# Autodesk Inventor assembly: BaseBoard
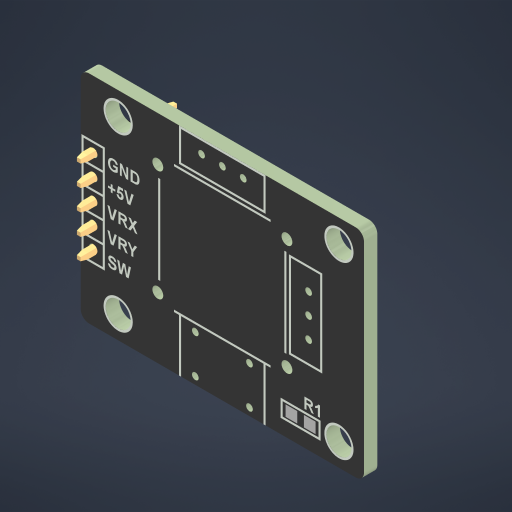
[picture p0: Inventor's stored thumbnail of the model, 512x512]
Saved by Autodesk Inventor 2024 (Build 280153000, 153)
## iProperties
Created: 2025-11-30
Part Number: BaseBoard
Document SubType Name: Assembly
Designer: Vincent Larson
Author: Vincent Larson
## Documents named in this file (3)
- C:\Users\Vincent Larson\Downloads\Digital Ship Challenge\Digital Ship Challenge Remote\KY-023_Joystick-Module\BaseBoard.iam
- C:\Users\Vincent Larson\Downloads\Digital Ship Challenge\Digital Ship Challenge Remote\KY-023_Joystick-Module\PCB.ipt
- C:\Users\Vincent Larson\Downloads\Digital Ship Challenge\Digital Ship Challenge Remote\Pin Headers\5 pin header.iam
## Components (2 placed, 2 different names)
1. 7 — Mate:1
2. 5 pin header:1 [sub-assembly] — Mate:1
## Relationships (1: Mate 1)
- Mate:1: 7 ↔ 5 pin header:1
